# Autodesk Inventor assembly: Mixing_Hotend
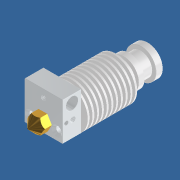
[picture p0: Inventor's stored thumbnail of the model, 180x180]
Saved by Autodesk Inventor 2020 (Build 240168000, 168)
## iProperties
Created: 2021-05-06
Part Number: Mixing_Hotend
Document SubType Name: Assembly
Designer: ken113
Author: ken113
## Documents named in this file (4)
- D:\Document\Github\Cheap_Belt_Printer\Model\Parts\Hotend\Mixing_Hotend\Mixing_Hotend.iam
- D:\Document\Github\Cheap_Belt_Printer\Model\Parts\Hotend\Mixing_Hotend\Heat_Block.ipt
- D:\Document\Github\Cheap_Belt_Printer\Model\Parts\Hotend\mk8-nozzle-0-4mm-2.snapshot.1\MK8 nozzle 0,4mm.ipt
- D:\Document\Github\Cheap_Belt_Printer\Model\Parts\Hotend\E3D_V6\e3dv6-full-complete-hotend-assembly-1.snapshot.2\E3Dv6 Full -Half_Hotend.iam
## Components (3 placed, 3 different names)
1. Heat_Block:1 — 挿入:1
2. Сопло MK8:1 — 挿入:2
3. E3Dv6 Full -Half_Hotend:1 [sub-assembly] — 挿入:1, 挿入:2
## Relationships (2: Insert 2)
- 挿入:1 [Insert]: Heat_Block:1 ↔ E3Dv6 Full -Half_Hotend:1
- 挿入:2 [Insert]: Сопло MK8:1 ↔ E3Dv6 Full -Half_Hotend:1
